# Autodesk Inventor assembly: Montagem2
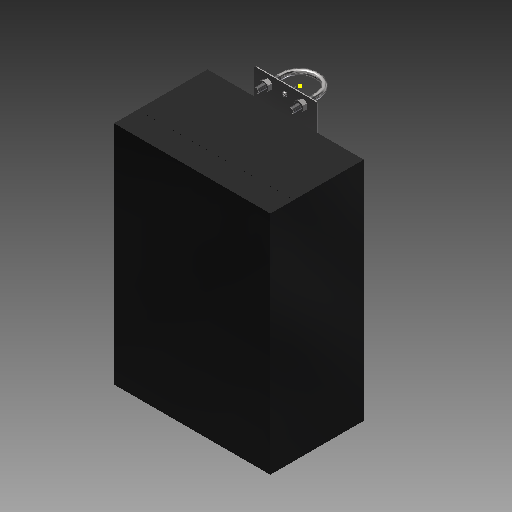
[picture p0: Inventor's stored thumbnail of the model, 512x512]
Saved by Autodesk Inventor 2019.4 (Build 234330000, 330)
## iProperties
Created: 2020-12-12
Part Number: Montagem2
Material: Genérico
Document SubType Name: Assembly
Designer: Lattes
Author: Lattes
## Documents named in this file (21)
- D:\Lattes\Documents\GitHub-HD\estacao-meteorologica-it\Estuturas\estrutura_telhado\caixa\caixa de instrumentação e controle.iam
- D:\Lattes\Documents\GitHub-HD\estacao-meteorologica-it\Estuturas\estrutura_telhado\caixa\base da caixa.ipt
- D:\Lattes\Documents\GitHub-HD\estacao-meteorologica-it\Estuturas\estrutura_telhado\caixa\fixador bateria v2.5.ipt
- D:\Lattes\Documents\GitHub-HD\estacao-meteorologica-it\Estuturas\estrutura_telhado\caixa\bateria 12mva-7.ipt
- D:\Lattes\Documents\GitHub-HD\estacao-meteorologica-it\Estuturas\estrutura_telhado\caixa\fixador bateria v2.5 - L.ipt
- D:\Lattes\Documents\GitHub-HD\estacao-meteorologica-it\Estuturas\estrutura_telhado\caixa\controlador solar v1.ipt
- D:\Lattes\Documents\GitHub-HD\estacao-meteorologica-it\Estuturas\estrutura_telhado\caixa\encaixe suporte controlador L.ipt
- D:\Lattes\Documents\GitHub-HD\estacao-meteorologica-it\Estuturas\estrutura_telhado\caixa\respirador_v1.ipt
- D:\Lattes\Documents\GitHub-HD\estacao-meteorologica-it\Estuturas\estrutura_telhado\caixa\borracha isolamento respirador.ipt
- D:\Lattes\Documents\GitHub-HD\estacao-meteorologica-it\Estuturas\estrutura_telhado\caixa\Parafuso m3 15mm.ipt
- D:\Lattes\Documents\GitHub-HD\estacao-meteorologica-it\Estuturas\estrutura_telhado\caixa\porca m3.ipt
- D:\Lattes\Documents\GitHub-HD\estacao-meteorologica-it\Estuturas\estrutura_telhado\caixa\borracha isolamento prensa cabo.ipt
- D:\Lattes\Documents\GitHub-HD\estacao-meteorologica-it\Estuturas\estrutura_telhado\caixa\prensa_cabo_fixador.ipt
- D:\Lattes\Documents\GitHub-HD\estacao-meteorologica-it\Estuturas\estrutura_telhado\caixa\chapa-fixação-caixa.ipt
- D:\Lattes\Documents\GitHub-HD\estacao-meteorologica-it\Estuturas\estrutura_telhado\caixa\ruela m6 borracha.ipt
- D:\Lattes\Documents\GitHub-HD\estacao-meteorologica-it\Estuturas\estrutura_telhado\caixa\parafuso-m6.ipt
- D:\Lattes\Documents\GitHub-HD\estacao-meteorologica-it\Estuturas\estrutura_telhado\caixa\ruela m6.ipt
- D:\Lattes\Documents\GitHub-HD\estacao-meteorologica-it\Estuturas\estrutura_telhado\caixa\porca m6.ipt
- D:\Lattes\Documents\GitHub-HD\estacao-meteorologica-it\Estuturas\estrutura_telhado\caixa\parafuso u abraçadeira menor.ipt
- D:\Lattes\Documents\GitHub-HD\estacao-meteorologica-it\Estuturas\estrutura_telhado\caixa\tampa caixa.ipt
- D:\Lattes\Documents\GitHub-HD\estacao-meteorologica-it\Estuturas\estrutura_telhado\caixa\espaçador 15mm m3.ipt
## Components (45 placed, 20 different names)
1. base da caixa:1 — Inserir:1, Coincidência:3, Coincidência:4, Inserir:2, Inserir:4, Inserir:6, Inserir:7, Inserir:8, Inserir:12, Inserir:13, Inserir:20, Inserir:21, Inserir:22, Inserir:23, Inserir:40, Inserir:41, Inserir:70, Inserir:71, Coincidência:7, Coincidência:8, Inserir:81, Inserir:82, Inserir:83
2. fixador bateria v2.5:1 — Inserir:1, Coincidência:1, Coincidência:2, Tangente:1, Coincidência:5, Coincidência:6
3. bateria 12mva-7:1 — Coincidência:1, Coincidência:2, Coincidência:3, Coincidência:4
4. fixador bateria v2.5 - L:1 — Inserir:2, Inserir:3
5. controlador solar v1:1 — Tangente:1, Coincidência:5, Coincidência:6
6. encaixe suporte controlador L:1 — Inserir:3
7. respirador_v1:1 — Inserir:4, Inserir:5, Inserir:9, Inserir:10, Inserir:11
8. borracha isolamento respirador:1 — Inserir:5
9. Parafuso m3 15mm:1 — Inserir:6
10. Parafuso m3 15mm:2 — Inserir:8
11. Parafuso m3 15mm:3 — Inserir:7
12. porca m3:1 — Inserir:9
13. porca m3:2 — Inserir:11
14. porca m3:3 — Inserir:10
15. borracha isolamento prensa cabo:1 — Inserir:12, Inserir:14
16. borracha isolamento prensa cabo:2 — Inserir:13, Inserir:15
17. prensa_cabo_fixador:1 — Inserir:14, Inserir:18, Inserir:19
18. prensa_cabo_fixador:2 — Inserir:15, Inserir:16, Inserir:17
19. Parafuso m3 15mm:4 — Inserir:18
20. porca m3:4 — Inserir:22
21. Parafuso m3 15mm:5 — Inserir:19
22. porca m3:5 — Inserir:23
23. Parafuso m3 15mm:6 — Inserir:17
24. porca m3:6 — Inserir:21
25. Parafuso m3 15mm:7 — Inserir:16
26. porca m3:7 — Inserir:20
27. ruela m6 borracha:3 — Inserir:34, Inserir:69
28. ruela m6 borracha:4 — Inserir:35, Inserir:68
29. parafuso-m6:3 — Inserir:35
30. parafuso-m6:4 — Inserir:34
31. ruela m6 borracha:5 — Inserir:43
32. ruela m6 borracha:8 — Inserir:42, Inserir:49
33. ruela m6:1 — Inserir:41, Inserir:43, Inserir:48
34. ruela m6:2 — Inserir:40, Inserir:42
35. porca m6:3 — Inserir:49
36. porca m6:4 — Inserir:48
37. porca m6:5 — Inserir:67
38. porca m6:6 — Inserir:66
39. chapa-fixação-caixa:1 — Inserir:66, Inserir:67, Inserir:68, Inserir:69, Inserir:70, Inserir:71, Inserir:79, Inserir:80
40. parafuso u abraçadeira menor:1 — Inserir:79
41. Parafuso m3 15mm:8 — Inserir:80
42. tampa caixa:2 — Coincidência:7, Coincidência:8
43. espaçador 15mm m3:1 — Inserir:81
44. espaçador 15mm m3:2 — Inserir:82
45. espaçador 15mm m3:3 — Inserir:83
## Relationships (51: Insert 42, Mate 8, Tangent 1)
- Inserir:1 (-5 mm): base da caixa:1 ↔ fixador bateria v2.5:1
- Coincidência:1 [Mate] (1 mm): fixador bateria v2.5:1 ↔ bateria 12mva-7:1
- Coincidência:2 [Mate]: fixador bateria v2.5:1 ↔ bateria 12mva-7:1
- Coincidência:3 [Mate] (1 mm): base da caixa:1 ↔ bateria 12mva-7:1
- Coincidência:4 [Mate] (0.5 mm): base da caixa:1 ↔ bateria 12mva-7:1
- Inserir:2: base da caixa:1 ↔ fixador bateria v2.5 - L:1
- Tangente:1: fixador bateria v2.5:1 ↔ controlador solar v1:1
- Coincidência:5 [Mate]: fixador bateria v2.5:1 ↔ controlador solar v1:1
- Inserir:3 (-3 mm): fixador bateria v2.5 - L:1 ↔ encaixe suporte controlador L:1
- Coincidência:6 [Mate]: fixador bateria v2.5:1 ↔ controlador solar v1:1
- Inserir:4 (1 mm): base da caixa:1 ↔ respirador_v1:1
- Inserir:5: respirador_v1:1 ↔ borracha isolamento respirador:1
- Inserir:6: base da caixa:1 ↔ Parafuso m3 15mm:1
- Inserir:7: base da caixa:1 ↔ Parafuso m3 15mm:3
- Inserir:8: base da caixa:1 ↔ Parafuso m3 15mm:2
- Inserir:9: respirador_v1:1 ↔ porca m3:1
- Inserir:10: respirador_v1:1 ↔ porca m3:3
- Inserir:11: respirador_v1:1 ↔ porca m3:2
- Inserir:12: base da caixa:1 ↔ borracha isolamento prensa cabo:1
- Inserir:13: base da caixa:1 ↔ borracha isolamento prensa cabo:2
- Inserir:14: borracha isolamento prensa cabo:1 ↔ prensa_cabo_fixador:1
- Inserir:15: borracha isolamento prensa cabo:2 ↔ prensa_cabo_fixador:2
- Inserir:16: prensa_cabo_fixador:2 ↔ Parafuso m3 15mm:7
- Inserir:17: prensa_cabo_fixador:2 ↔ Parafuso m3 15mm:6
- Inserir:18: prensa_cabo_fixador:1 ↔ Parafuso m3 15mm:4
- Inserir:19: prensa_cabo_fixador:1 ↔ Parafuso m3 15mm:5
- Inserir:20: base da caixa:1 ↔ porca m3:7
- Inserir:21: base da caixa:1 ↔ porca m3:6
- Inserir:22: base da caixa:1 ↔ porca m3:4
- Inserir:23: base da caixa:1 ↔ porca m3:5
- Inserir:34: ruela m6 borracha:3 ↔ parafuso-m6:4
- Inserir:35: ruela m6 borracha:4 ↔ parafuso-m6:3
- Inserir:40: base da caixa:1 ↔ ruela m6:2
- Inserir:41: base da caixa:1 ↔ ruela m6:1
- Inserir:42: ruela m6 borracha:8 ↔ ruela m6:2
- Inserir:43: ruela m6 borracha:5 ↔ ruela m6:1
- Inserir:48: ruela m6:1 ↔ porca m6:4
- Inserir:49: ruela m6 borracha:8 ↔ porca m6:3
- Inserir:66: porca m6:6 ↔ chapa-fixação-caixa:1
- Inserir:67: porca m6:5 ↔ chapa-fixação-caixa:1
- Inserir:68: ruela m6 borracha:4 ↔ chapa-fixação-caixa:1
- Inserir:69: ruela m6 borracha:3 ↔ chapa-fixação-caixa:1
- Inserir:70: base da caixa:1 ↔ chapa-fixação-caixa:1
- Inserir:71: base da caixa:1 ↔ chapa-fixação-caixa:1
- Inserir:79 (-14.5 mm): chapa-fixação-caixa:1 ↔ parafuso u abraçadeira menor:1
- Inserir:80: chapa-fixação-caixa:1 ↔ Parafuso m3 15mm:8
- Coincidência:7 [Mate]: base da caixa:1 ↔ tampa caixa:2
- Coincidência:8 [Mate]: base da caixa:1 ↔ tampa caixa:2
- Inserir:81: base da caixa:1 ↔ espaçador 15mm m3:1
- Inserir:82: base da caixa:1 ↔ espaçador 15mm m3:2
- Inserir:83: base da caixa:1 ↔ espaçador 15mm m3:3
